# Autodesk Inventor assembly: RFID
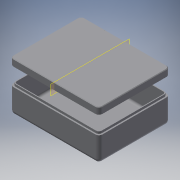
[picture p0: Inventor's stored thumbnail of the model, 180x180]
Saved by Autodesk Inventor 2016 (Build 200138000, 138)
## iProperties
Created: 2015-10-01
Part Number: RFID
Document SubType Name: Assembly
Designer: Drew
Author: Drew
## Documents named in this file (3)
- C:\Users\Drew\Documents\Soapy CAD\RFID.iam
- C:\Users\Drew\Documents\Soapy CAD\RFID_Box.ipt
- C:\Users\Drew\Documents\Soapy CAD\RFID_Lid.ipt
## Components (2 placed, 2 different names)
1. RFID_Lid:1 — Flush:1, Flush:2
2. RFID_Box:1 — Flush:1, Flush:2
## Relationships (2: Flush 2)
- Flush:1: RFID_Lid:1 ↔ RFID_Box:1
- Flush:2: RFID_Lid:1 ↔ RFID_Box:1
